# Autodesk Inventor assembly: SDS MK4i Swerve Module NEOS_Harnessed
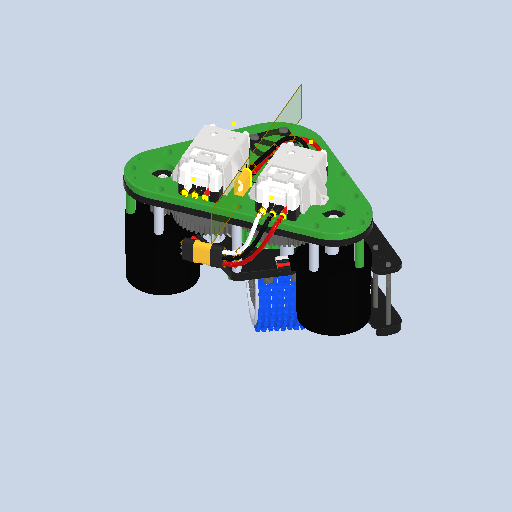
[picture p0: Inventor's stored thumbnail of the model, 512x512]
Saved by Autodesk Inventor 2023.3 (Build 273359000, 359)
## iProperties
Created: 2023-03-28
Part Number: SDS MK4i Swerve Module NEOS_Harnessed
Document SubType Name: Assembly
Designer: jackc
Author: jackc
## Documents named in this file (10)
- D:\.shortcut-targets-by-id\104lhnwPhYvankLacu8RGROV89Bx_24Mg\1939\2_Design\2023-2024\Parts\Swerve\SDS MK4i Swerve Module NEOS_Harnessed.iam
- D:\.shortcut-targets-by-id\104lhnwPhYvankLacu8RGROV89Bx_24Mg\1939\2_Design\2023-2024\Parts\Swerve\NEO Drive Gear.iam
- D:\.shortcut-targets-by-id\104lhnwPhYvankLacu8RGROV89Bx_24Mg\1939\2_Design\2023-2024\Parts\Swerve\NEO Turn Gear.iam
- D:\.shortcut-targets-by-id\104lhnwPhYvankLacu8RGROV89Bx_24Mg\1939\2_Design\2023-2024\Parts\Swerve\SDS MK4i Swerve Module, unpopulated.iam
- D:\.shortcut-targets-by-id\104lhnwPhYvankLacu8RGROV89Bx_24Mg\1939\2_Design\2023-2024\Parts\Motors\NEO Motor.ipt
- D:\.shortcut-targets-by-id\104lhnwPhYvankLacu8RGROV89Bx_24Mg\1939\2_Design\2023-2024\Parts\Printed Parts\Module_SPM_Mount.ipt
- D:\.shortcut-targets-by-id\104lhnwPhYvankLacu8RGROV89Bx_24Mg\1939\2_Design\2023-2024\Parts\Electronics\Motor Controllers\REV-11-2158-Spark-MAX.ipt
- D:\.shortcut-targets-by-id\104lhnwPhYvankLacu8RGROV89Bx_24Mg\1939\2_Design\2023-2024\Parts\Electronics\Motor Controllers\REV-21-2151_SPM_Mount.ipt
- D:\.shortcut-targets-by-id\104lhnwPhYvankLacu8RGROV89Bx_24Mg\1939\2_Design\2023-2024\Parts\Electronics\Motor Controllers\SpMax_Drive.iam
- D:\.shortcut-targets-by-id\104lhnwPhYvankLacu8RGROV89Bx_24Mg\1939\2_Design\2023-2024\Parts\Electronics\Connectors\MR60_Recp.iam
## Components (11 placed, 9 different names)
1. NEO Drive Gear:1 [sub-assembly]
2. NEO Turn Gear:1 [sub-assembly]
3. SDS MK4i Swerve Module, unpopulated:1 [sub-assembly] — Mate:13, Mate:14, Mate:15, Mate:16, Mate:17, Mate:18
4. NEO Motor:1 — Mate:13, Mate:14, Mate:15
5. NEO Motor:2 — Mate:16, Mate:17, Mate:18
6. Module_SPM_Mount:1 — Mate:7, Flush:1, Mate:19, Flush:23
7. SpMax_Drive:1 [sub-assembly] — Mate:7, Flush:1, Mate:10, Angle:3, Symmetry:1
8. REV-11-2158-Spark-MAX:2 — Symmetry:1
9. REV-21-2151_SPM_Mount:1
10. REV-21-2151_SPM_Mount:2 — Mate:10, Angle:3
11. MR60_Recp:1 [sub-assembly] — Mate:19, Flush:23, Flush:22
## Relationships (28: Mate 19, Angle 4, Flush 3, Tangent 1, Symmetry 1)
- [Mate]: SDS MK4i Swerve Module, unpopulated:1 ↔ Module_SPM_Mount:1
- [Mate]: SDS MK4i Swerve Module, unpopulated:1 ↔ Module_SPM_Mount:1
- [Mate]: SDS MK4i Swerve Module, unpopulated:1 ↔ Module_SPM_Mount:1
- [Mate]: SDS MK4i Swerve Module, unpopulated:1 ↔ Module_SPM_Mount:1
- [Angle] (180 deg): SDS MK4i Swerve Module, unpopulated:1 ↔ Module_SPM_Mount:1
- [Mate]: SDS MK4i Swerve Module, unpopulated:1 ↔ Module_SPM_Mount:1
- [Mate]: Module_SPM_Mount:1 ↔ REV-11-2158-Spark-MAX:2
- Mate:7: Module_SPM_Mount:1 ↔ SpMax_Drive:1
- Flush:1 (5.08 mm): Module_SPM_Mount:1 ↔ SpMax_Drive:1
- [Mate]: REV-11-2158-Spark-MAX:2 ↔ REV-21-2151_SPM_Mount:1
- [Angle] (0 deg): REV-11-2158-Spark-MAX:2 ↔ REV-21-2151_SPM_Mount:1
- [Mate]: Module_SPM_Mount:1 ↔ REV-21-2151_SPM_Mount:1
- Mate:10: SpMax_Drive:1 ↔ REV-21-2151_SPM_Mount:2
- Angle:3 (0 deg): SpMax_Drive:1 ↔ REV-21-2151_SPM_Mount:2
- [Mate]: Module_SPM_Mount:1 ↔ REV-21-2151_SPM_Mount:2
- [Tangent] (4.445 mm): SDS MK4i Swerve Module, unpopulated:1 ↔ REV-21-2151_SPM_Mount:2
- [Mate]: Module_SPM_Mount:1 ↔ REV-21-2151_SPM_Mount:1
- [Angle] (90 deg): Module_SPM_Mount:1 ↔ REV-11-2158-Spark-MAX:2
- Mate:13: SDS MK4i Swerve Module, unpopulated:1 ↔ NEO Motor:1
- Mate:14: SDS MK4i Swerve Module, unpopulated:1 ↔ NEO Motor:1
- Mate:15: SDS MK4i Swerve Module, unpopulated:1 ↔ NEO Motor:1
- Mate:16: SDS MK4i Swerve Module, unpopulated:1 ↔ NEO Motor:2
- Mate:17: SDS MK4i Swerve Module, unpopulated:1 ↔ NEO Motor:2
- Mate:18: SDS MK4i Swerve Module, unpopulated:1 ↔ NEO Motor:2
- Mate:19 (6.35 mm): Module_SPM_Mount:1 ↔ MR60_Recp:1
- Flush:23 (38.1 mm): Module_SPM_Mount:1 ↔ MR60_Recp:1
- Symmetry:1: SpMax_Drive:1 ↔ REV-11-2158-Spark-MAX:2
- Flush:22 (-25.4 mm): MR60_Recp:1
